# Autodesk Inventor assembly: Gaveta
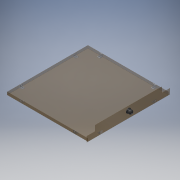
[picture p0: Inventor's stored thumbnail of the model, 180x180]
Saved by Autodesk Inventor 2018 (Build 220112000, 112)
## iProperties
Created: 2018-07-08
Part Number: Gaveta
Material: Genérico
Document SubType Name: Assembly
Designer: Regner
Author: Regner
## Documents named in this file (8)
- C:\Users\Regner\Documents\ROBOTA\2018\Tortura Ratos\Gaveta.iam
- C:\Users\Regner\Documents\ROBOTA\2018\Tortura Ratos\Tampa Gaveta.ipt
- C:\Users\Regner\Documents\ROBOTA\2018\Tortura Ratos\Fundo Gaveta.ipt
- C:\Users\Regner\Documents\ROBOTA\2018\Tortura Ratos\Lateral 1 Gaveta.ipt
- C:\Users\Regner\Documents\ROBOTA\2018\Tortura Ratos\Lateral 2 Gaveta.ipt
- C:\Users\Regner\Documents\ROBOTA\2018\Tortura Ratos\Cantoneira Gaveta.ipt
- C:\Users\Regner\Documents\ROBOTA\2018\Tortura Ratos\Puxador.ipt
- C:\Users\Regner\Documents\Inventor\Content Center Files\R2018\pt-BR\GB_T 822-2000 H\Screw GB_T 822 M2 x 8.ipt
## Components (15 placed, 7 different names)
1. Tampa Gaveta:1 — Coincidência:1, Alinhamento:1, Alinhamento:2, Coincidência:5, Coincidência:6, Coincidência:31, Coincidência:32, Coincidência:33, Coincidência:34, Coincidência:36
2. Fundo Gaveta:1 — Coincidência:1, Alinhamento:1, Alinhamento:2, Coincidência:2, Alinhamento:3, Alinhamento:4, Coincidência:3, Coincidência:4, Alinhamento:5, Alinhamento:6, Coincidência:7, Coincidência:8, Coincidência:9, Coincidência:10, Coincidência:11, Coincidência:12, Coincidência:13, Coincidência:14, Coincidência:15, Coincidência:16, Coincidência:17, Coincidência:18, Coincidência:19, Coincidência:20, Coincidência:21, Coincidência:27, Alinhamento:7, Alinhamento:8, Alinhamento:9
3. Lateral 1 Gaveta:1 — Coincidência:2, Alinhamento:3, Alinhamento:4, Coincidência:22, Coincidência:23, Coincidência:24, Coincidência:29
4. Lateral 2 Gaveta:1 — Coincidência:4, Coincidência:5, Alinhamento:5, Coincidência:25, Coincidência:30
5. Lateral 2 Gaveta:2 — Coincidência:3, Coincidência:6, Alinhamento:6, Coincidência:26, Coincidência:28
6. Cantoneira Gaveta:1 — Coincidência:8, Coincidência:20, Coincidência:22, Coincidência:29
7. Cantoneira Gaveta:2 — Coincidência:12, Coincidência:17, Coincidência:30
8. Cantoneira Gaveta:3 — Coincidência:10, Coincidência:26, Coincidência:27
9. Cantoneira Gaveta:4 — Coincidência:9, Coincidência:21, Coincidência:28
10. Cantoneira Gaveta:5 — Coincidência:13, Coincidência:16, Coincidência:31
11. Cantoneira Gaveta:6 — Coincidência:14, Coincidência:15, Coincidência:32
12. Cantoneira Gaveta:9 — Coincidência:11, Coincidência:19, Coincidência:25
13. Cantoneira Gaveta:10 — Coincidência:7, Coincidência:18, Coincidência:23, Coincidência:24
14. Puxador:1 — Coincidência:33, Coincidência:34, Coincidência:35
15. Screw GB/T 822-2000 Type H M2 x 8:1 — Coincidência:35, Coincidência:36
## Relationships (45: Mate 36, Flush 9)
- Coincidência:1 [Mate]: Tampa Gaveta:1 ↔ Fundo Gaveta:1
- Alinhamento:1 [Flush]: Tampa Gaveta:1 ↔ Fundo Gaveta:1
- Alinhamento:2 [Flush] (4.4 mm): Tampa Gaveta:1 ↔ Fundo Gaveta:1
- Coincidência:2 [Mate]: Fundo Gaveta:1 ↔ Lateral 1 Gaveta:1
- Alinhamento:3 [Flush]: Fundo Gaveta:1 ↔ Lateral 1 Gaveta:1
- Alinhamento:4 [Flush]: Fundo Gaveta:1 ↔ Lateral 1 Gaveta:1
- Coincidência:3 [Mate]: Fundo Gaveta:1 ↔ Lateral 2 Gaveta:2
- Coincidência:4 [Mate]: Fundo Gaveta:1 ↔ Lateral 2 Gaveta:1
- Coincidência:5 [Mate]: Tampa Gaveta:1 ↔ Lateral 2 Gaveta:1
- Coincidência:6 [Mate]: Tampa Gaveta:1 ↔ Lateral 2 Gaveta:2
- Alinhamento:5 [Flush]: Fundo Gaveta:1 ↔ Lateral 2 Gaveta:1
- Alinhamento:6 [Flush]: Fundo Gaveta:1 ↔ Lateral 2 Gaveta:2
- Coincidência:7 [Mate]: Fundo Gaveta:1 ↔ Cantoneira Gaveta:10
- Coincidência:8 [Mate]: Fundo Gaveta:1 ↔ Cantoneira Gaveta:1
- Coincidência:9 [Mate]: Fundo Gaveta:1 ↔ Cantoneira Gaveta:4
- Coincidência:10 [Mate]: Fundo Gaveta:1 ↔ Cantoneira Gaveta:3
- Coincidência:11 [Mate]: Fundo Gaveta:1 ↔ Cantoneira Gaveta:9
- Coincidência:12 [Mate]: Fundo Gaveta:1 ↔ Cantoneira Gaveta:2
- Coincidência:13 [Mate]: Fundo Gaveta:1 ↔ Cantoneira Gaveta:5
- Coincidência:14 [Mate]: Fundo Gaveta:1 ↔ Cantoneira Gaveta:6
- Coincidência:15 [Mate]: Fundo Gaveta:1 ↔ Cantoneira Gaveta:6
- Coincidência:16 [Mate]: Fundo Gaveta:1 ↔ Cantoneira Gaveta:5
- Coincidência:17 [Mate]: Fundo Gaveta:1 ↔ Cantoneira Gaveta:2
- Coincidência:18 [Mate]: Fundo Gaveta:1 ↔ Cantoneira Gaveta:10
- Coincidência:19 [Mate]: Fundo Gaveta:1 ↔ Cantoneira Gaveta:9
- Coincidência:20 [Mate]: Fundo Gaveta:1 ↔ Cantoneira Gaveta:1
- Coincidência:21 [Mate]: Fundo Gaveta:1 ↔ Cantoneira Gaveta:4
- Coincidência:22 [Mate]: Lateral 1 Gaveta:1 ↔ Cantoneira Gaveta:1
- Coincidência:23 [Mate]: Lateral 1 Gaveta:1 ↔ Cantoneira Gaveta:10
- Coincidência:24 [Mate]: Lateral 1 Gaveta:1 ↔ Cantoneira Gaveta:10
- Coincidência:25 [Mate]: Lateral 2 Gaveta:1 ↔ Cantoneira Gaveta:9
- Coincidência:26 [Mate]: Lateral 2 Gaveta:2 ↔ Cantoneira Gaveta:3
- Coincidência:27 [Mate]: Fundo Gaveta:1 ↔ Cantoneira Gaveta:3
- Coincidência:28 [Mate]: Lateral 2 Gaveta:2 ↔ Cantoneira Gaveta:4
- Coincidência:29 [Mate]: Lateral 1 Gaveta:1 ↔ Cantoneira Gaveta:1
- Coincidência:30 [Mate]: Lateral 2 Gaveta:1 ↔ Cantoneira Gaveta:2
- Coincidência:31 [Mate]: Tampa Gaveta:1 ↔ Cantoneira Gaveta:5
- Coincidência:32 [Mate]: Tampa Gaveta:1 ↔ Cantoneira Gaveta:6
- Coincidência:33 [Mate]: Tampa Gaveta:1 ↔ Puxador:1
- Coincidência:34 [Mate]: Tampa Gaveta:1 ↔ Puxador:1
- Alinhamento:7 [Flush]: Fundo Gaveta:1
- Alinhamento:8 [Flush]: Fundo Gaveta:1
- Alinhamento:9 [Flush]: Fundo Gaveta:1
- Coincidência:35 [Mate]: Puxador:1 ↔ Screw GB/T 822-2000 Type H M2 x 8:1
- Coincidência:36 [Mate]: Tampa Gaveta:1 ↔ Screw GB/T 822-2000 Type H M2 x 8:1
